# Autodesk Inventor assembly: varsity wheel with sprocket
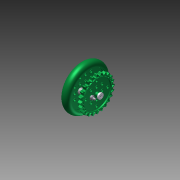
[picture p0: Inventor's stored thumbnail of the model, 180x180]
Saved by Autodesk Inventor 2014 SP1 (Build 180222100, 222)
## iProperties
Created: 2014-02-23
Part Number: varsity wheel with sprocket
Document SubType Name: Assembly
Designer: Ryan
Author: Ryan
## Documents named in this file (10)
- C:\Users\Ryan\Desktop\sw\toss up 5th A bot\drive\varsity wheel with sprocket.iam
- C:\Users\Ryan\Desktop\sw\toss up 4th robot\drive\varsity wheel.iam
- C:\Users\Ryan\Desktop\sw\lib\Aperture VEX CAD Library\Sprockets\green\High Strength 24-Tooth Sprocket.ipt
- C:\Users\Ryan\Desktop\sw\lib\Aperture VEX CAD Library\Hardware\8-32\8-32_1.500.ipt
- C:\Users\Ryan\Desktop\sw\lib\Aperture VEX CAD Library\Spacers\SPACER-0500-0250.ipt
- C:\Users\Ryan\Desktop\sw\lib\Aperture VEX CAD Library\Hardware\8-32\8-32 nylock.ipt
- C:\Users\Ryan\Desktop\sw\lib\Aperture VEX CAD Library\Spacers\SPACER-0500-0125.ipt
- C:\Users\Ryan\Desktop\sw\lib\Aperture VEX CAD Library\Spacers\SPACER-0500-0375.ipt
- C:\Users\Ryan\Desktop\sw\lib\Aperture VEX CAD Library\Spacers\SPACER-0500-0500.ipt
- C:\Users\Ryan\Desktop\sw\lib\Aperture VEX CAD Library\Shaft\2 inch Shaft.ipt
## Components (14 placed, 9 different names)
1. varsity wheel:1 [sub-assembly] — Mate:1, Mate:2, Mate:3, Mate:10, Mate:11, Mate:16, Flush:21, Mate:20, Mate:21
2. High Strength 24-Tooth Sprocket:1 — Mate:1, Mate:2, Mate:3, Mate:9, Mate:12, Mate:13, Mate:22
3. SPACER-0500-0250:2 — Mate:10, Mate:11, Mate:14, Mate:15
4. SPACER-0500-0125:1 — Mate:12, Mate:13
5. SPACER-0500-0125:2 — Mate:14, Mate:15
6. 2 inch Shaft:1 — Flush:21, Mate:20, Mate:21
7. 8-32_1.500:1 — Mate:8, Mate:17, Mate:18, Mate:22
8. 8-32 nylock:1 — Mate:8, Mate:9
9. SPACER-0500-0500:1 — Mate:18, Mate:19
10. SPACER-0500-0375:1 — Mate:16, Mate:17, Mate:19
11. 8-32_1.500:2
12. 8-32 nylock:2
13. SPACER-0500-0500:2
14. SPACER-0500-0375:2
## Component patterns: (2 elements, first: 8-32_1.500:1 + 8-32 nylock:1 + SPACER-0500-0500:1 + SPACER-0500-0375:1)
## Relationships (20: Mate 19, Flush 1)
- Mate:1: varsity wheel:1 ↔ High Strength 24-Tooth Sprocket:1
- Mate:2: varsity wheel:1 ↔ High Strength 24-Tooth Sprocket:1
- Mate:3 (9.525 mm): varsity wheel:1 ↔ High Strength 24-Tooth Sprocket:1
- [Mate]: varsity wheel:1 ↔ 8-32_1.500:1
- Mate:8: 8-32_1.500:1 ↔ 8-32 nylock:1
- Mate:9: High Strength 24-Tooth Sprocket:1 ↔ 8-32 nylock:1
- Mate:10: varsity wheel:1 ↔ SPACER-0500-0250:2
- Mate:11: varsity wheel:1 ↔ SPACER-0500-0250:2
- Mate:12: High Strength 24-Tooth Sprocket:1 ↔ SPACER-0500-0125:1
- Mate:13: High Strength 24-Tooth Sprocket:1 ↔ SPACER-0500-0125:1
- Mate:14: SPACER-0500-0250:2 ↔ SPACER-0500-0125:2
- Mate:15: SPACER-0500-0250:2 ↔ SPACER-0500-0125:2
- Mate:16: varsity wheel:1 ↔ SPACER-0500-0375:1
- Mate:17: 8-32_1.500:1 ↔ SPACER-0500-0375:1
- Mate:18: 8-32_1.500:1 ↔ SPACER-0500-0500:1
- Mate:19: SPACER-0500-0500:1 ↔ SPACER-0500-0375:1
- Flush:21 (-6.35 mm): varsity wheel:1 ↔ 2 inch Shaft:1
- Mate:20: varsity wheel:1 ↔ 2 inch Shaft:1
- Mate:21: varsity wheel:1 ↔ 2 inch Shaft:1
- Mate:22: High Strength 24-Tooth Sprocket:1 ↔ 8-32_1.500:1
